# Autodesk Inventor assembly: LINK2
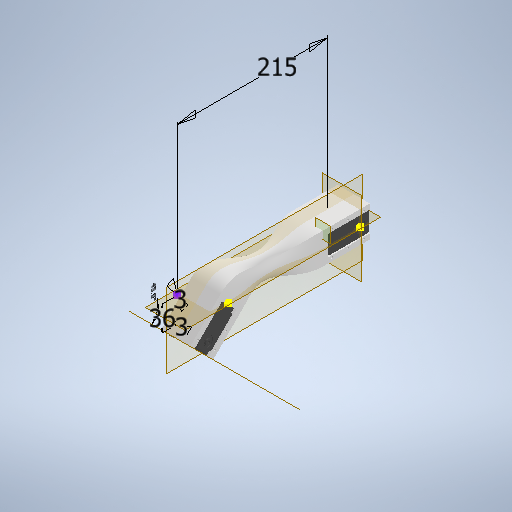
[picture p0: Inventor's stored thumbnail of the model, 512x512]
Saved by Autodesk Inventor 2026.1 (Build 301233020, 233B)
## iProperties
Created: 2025-10-15
Part Number: LINK2
Document SubType Name: Assembly
Designer: wlgns
Author: wlgns
## Documents named in this file (4)
- C:\Users\wlgns\Desktop\project\ARA Project\ARA_CAD_model\ARA_v2\LINK2.iam
- C:\Users\wlgns\Desktop\project\ARA Project\ARA_CAD_model\ARA_v2\ARM_1 SKETCH_smooth.ipt
- C:\Users\wlgns\Desktop\project\ARA Project\ARA_CAD_model\ARA_v2\MX-106T.ipt
- C:\Users\wlgns\Desktop\project\ARA Project\ARA_CAD_model\ARA_v2\MX-64R.ipt
## Components (3 placed, 3 different names)
1. ARM_1 SKETCH_smooth:1 — 메이트:1, 메이트:2, 플러쉬:1, 메이트:3, 메이트:5, 메이트:6, 각도:1, 메이트:7, 메이트:8, 메이트:9
2. MX-106T:1 — 메이트:1, 메이트:2, 플러쉬:1, 메이트:4
3. MX-64R:1 — 메이트:3, 메이트:5
## Relationships (11: Mate 9, Flush 1, Angle 1)
- 메이트:1 [Mate]: ARM_1 SKETCH_smooth:1 ↔ MX-106T:1
- 메이트:2 [Mate]: ARM_1 SKETCH_smooth:1 ↔ MX-106T:1
- 플러쉬:1 [Flush]: ARM_1 SKETCH_smooth:1 ↔ MX-106T:1
- 메이트:3 [Mate]: ARM_1 SKETCH_smooth:1 ↔ MX-64R:1
- 메이트:4 [Mate]: MX-106T:1
- 메이트:5 [Mate]: ARM_1 SKETCH_smooth:1 ↔ MX-64R:1
- 메이트:6 [Mate] (-23.2 mm): ARM_1 SKETCH_smooth:1
- 각도:1 [Angle] (180 deg): ARM_1 SKETCH_smooth:1
- 메이트:7 [Mate]: ARM_1 SKETCH_smooth:1
- 메이트:8 [Mate]: ARM_1 SKETCH_smooth:1
- 메이트:9 [Mate]: ARM_1 SKETCH_smooth:1
